# Autodesk Inventor assembly: New_Odom_Assembly
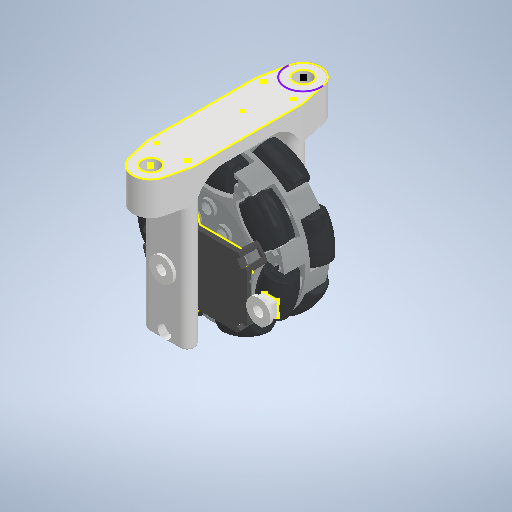
[picture p0: Inventor's stored thumbnail of the model, 512x512]
Saved by Autodesk Inventor 2025.1 (Build 291241020, 241B)
## iProperties
Created: 2024-11-18
Part Number: New_Odom_Assembly
Document SubType Name: Assembly
Designer: AtuStem
Author: AtuStem
## Documents named in this file (12)
- C:\Users\AtuStem\Documents\GitHub\ATUM-V5RC-High-Stakes-CAD\Odometers_Collin\New_Odom_Assembly.iam
- C:\Users\AtuStem\Documents\GitHub\ATUM-V5RC-High-Stakes-CAD\Odometers_Collin\IQ_OMNI.iam
- C:\Users\AtuStem\Documents\GitHub\ATUM-V5RC-High-Stakes-CAD\Odometers_Collin\Latest_Odom.ipt
- C:\Users\AtuStem\Documents\GitHub\ATUM-V5RC-High-Stakes-CAD\Odometers_Collin\Encoder_Base.ipt
- C:\Users\AtuStem\Documents\GitHub\ATUM-V5RC-High-Stakes-CAD\VEX-CAD-Inventor\Motion\Insert Circle.ipt
- C:\Users\AtuStem\Documents\GitHub\ATUM-V5RC-High-Stakes-CAD\VEX-CAD-Inventor\Motion\Shaft LS\Shaft LS\Shaft LS 2.0.ipt
- C:\Users\AtuStem\Documents\GitHub\ATUM-V5RC-High-Stakes-CAD\VEX-CAD-Inventor\Motion\Shaft LS\Shaft LS.ipt
- C:\Users\AtuStem\Documents\GitHub\ATUM-V5RC-High-Stakes-CAD\VEX-CAD-Inventor\Motion\Shaft LS\Shaft Collar ipts\Shaft Collar No Screw.ipt
- C:\Users\AtuStem\Documents\GitHub\ATUM-V5RC-High-Stakes-CAD\VEX-CAD-Inventor\Motion\Spacers\Washer Teflon\TWasher .375 OD x .03125.ipt
- C:\Users\AtuStem\Documents\GitHub\ATUM-V5RC-High-Stakes-CAD\VEX-CAD-Inventor\Motion\Spacers\Washer Teflon.ipt
- C:\Users\AtuStem\Documents\GitHub\ATUM-V5RC-High-Stakes-CAD\VEX-CAD-Inventor\Motion\Spacers\Spacer Nylon .375 OD\NSpacer .375 OD x .500.ipt
- C:\Users\AtuStem\Documents\GitHub\ATUM-V5RC-High-Stakes-CAD\VEX-CAD-Inventor\Motion\Spacers\Spacer Nylon .375 OD.ipt
## Components (10 placed, 8 different names)
1. Latest_Odom:1 — Mate:2, Mate:3, Mate:4, Mate:5, Mate:6, Mate:7, Mate:8, Mate:11
2. IQ_OMNI:1 [sub-assembly] — Mate:4
3. Encoder_Base:1 — Mate:2, Mate:3
4. Insert Circle:1 — Mate:5, Mate:6, Mate:9
5. Insert Circle:2 — Mate:7, Mate:8, Mate:10, Mate:12
6. Shaft LS 2.0:1 — Mate:9
7. Shaft Collar No Screw:1 — Mate:10, Mate:13, Mate:14, Mate:15
8. TWasher .375 OD x .03125:1 — Mate:11, Mate:12, Mate:13
9. NSpacer .375 OD x .500:1 — Mate:14, Mate:15
10. Insert Circle:3
## Relationships (14: Mate 14)
- Mate:2: Latest_Odom:1 ↔ Encoder_Base:1
- Mate:3: Latest_Odom:1 ↔ Encoder_Base:1
- Mate:4: Latest_Odom:1 ↔ IQ_OMNI:1
- Mate:5: Latest_Odom:1 ↔ Insert Circle:1
- Mate:6: Latest_Odom:1 ↔ Insert Circle:1
- Mate:7: Latest_Odom:1 ↔ Insert Circle:2
- Mate:8: Latest_Odom:1 ↔ Insert Circle:2
- Mate:9: Insert Circle:1 ↔ Shaft LS 2.0:1
- Mate:10: Insert Circle:2 ↔ Shaft Collar No Screw:1
- Mate:11: Latest_Odom:1 ↔ TWasher .375 OD x .03125:1
- Mate:12: Insert Circle:2 ↔ TWasher .375 OD x .03125:1
- Mate:13: Shaft Collar No Screw:1 ↔ TWasher .375 OD x .03125:1
- Mate:14: Shaft Collar No Screw:1 ↔ NSpacer .375 OD x .500:1
- Mate:15: Shaft Collar No Screw:1 ↔ NSpacer .375 OD x .500:1
